# Autodesk Inventor assembly: ASM_Micron_Rev_with_Jigs
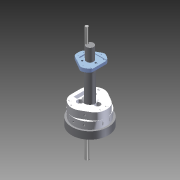
[picture p0: Inventor's stored thumbnail of the model, 180x180]
Saved by Autodesk Inventor 2011 SP2 (Build 150309200, 309)
## iProperties
Created: 2011-09-29
Part Number: ASM_Micron_Rev_with_Jigs
Document SubType Name: Assembly
Designer: sungwook
Author: sungwook
## Documents named in this file (7)
- C:\Users\sungwook\Documents\Inventor\Micron20\Assembly\ASM_Micron_Rev_with_Jigs.iam
- C:\Users\sungwook\Documents\Inventor\Micron20\Parts\Jigs\Jig_TopHeightAligner.ipt
- C:\Users\sungwook\Documents\Inventor\Micron20\Parts\Main\Platform_Base_20mm_Rev.ipt
- C:\Users\sungwook\Documents\Inventor\Micron20\Parts\Main\Platform_Top_14mm_Rev.ipt
- C:\Users\sungwook\Documents\Inventor\Micron20\Parts\Jigs\Jig_pin_p080.ipt
- C:\Users\sungwook\Documents\Inventor\Micron20\Parts\Jigs\Jig_pin_p118.ipt
- C:\Users\sungwook\Documents\Inventor\Micron20\Parts\Jigs\Jig_Aligner_Sleeve.ipt
## Components (6 placed, 6 different names)
1. Jig_TopHeightAligner:1 — Mate:1, Mate:5, Mate:6, Mate:7, Mate:11, Mate:12, Mate:9, Flush:15, Mate:15
2. Platform_Base_20mm_Rev:1 — Mate:1, Mate:10, Mate:12, Mate:14
3. Platform_Top_14mm_Rev:1 — Mate:5, Mate:6, Mate:7, Mate:8, Mate:16
4. Jig_pin_p080:1 — Mate:8, Mate:11
5. Jig_pin_p118:1 — Mate:9, Mate:10, Mate:14
6. Jig_Aligner_Sleeve:1 — Flush:15, Mate:15, Mate:16
## Relationships (13: Mate 12, Flush 1)
- Mate:1: Jig_TopHeightAligner:1 ↔ Platform_Base_20mm_Rev:1
- Mate:5: Jig_TopHeightAligner:1 ↔ Platform_Top_14mm_Rev:1
- Mate:6: Jig_TopHeightAligner:1 ↔ Platform_Top_14mm_Rev:1
- Mate:7: Jig_TopHeightAligner:1 ↔ Platform_Top_14mm_Rev:1
- Mate:8: Platform_Top_14mm_Rev:1 ↔ Jig_pin_p080:1
- Mate:9: Jig_TopHeightAligner:1 ↔ Jig_pin_p118:1
- Mate:10: Platform_Base_20mm_Rev:1 ↔ Jig_pin_p118:1
- Mate:11: Jig_TopHeightAligner:1 ↔ Jig_pin_p080:1
- Mate:12: Jig_TopHeightAligner:1 ↔ Platform_Base_20mm_Rev:1
- Mate:14: Platform_Base_20mm_Rev:1 ↔ Jig_pin_p118:1
- Flush:15 (-0.508 mm): Jig_TopHeightAligner:1 ↔ Jig_Aligner_Sleeve:1
- Mate:15: Jig_TopHeightAligner:1 ↔ Jig_Aligner_Sleeve:1
- Mate:16: Platform_Top_14mm_Rev:1 ↔ Jig_Aligner_Sleeve:1
